# Autodesk Inventor assembly: FlexCouplerAssembly
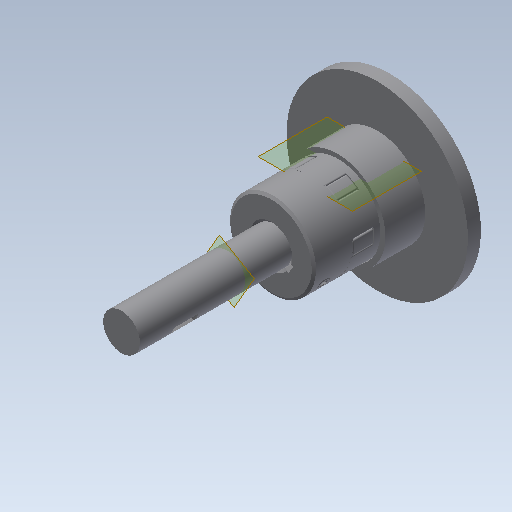
[picture p0: Inventor's stored thumbnail of the model, 512x512]
Saved by Autodesk Inventor 2021 (Build 250183000, 183)
## iProperties
Created: 2020-09-19
Part Number: FlexCouplerAssembly
Document SubType Name: Assembly
Designer: PhotonUser
Quantity: 1
Author: PhotonUser
## Documents named in this file (6)
- D:\PhotonUser\Downloads\Assembly Files-20201011T184130Z-001\Assembly Files\FlexCouplerAssembly.iam
- D:\PhotonUser\Downloads\Assembly Files-20201011T184130Z-001\Assembly Files\6408K139_FLEXIBLE SHAFT COUPLING ORIGINAL.ipt
- D:\PhotonUser\Downloads\Assembly Files-20201011T184130Z-001\Assembly Files\6408K139_FLEXIBLE SHAFT COUPLING.ipt
- D:\PhotonUser\Downloads\Assembly Files-20201011T184130Z-001\Assembly Files\6408K740_FLEXIBLE SHAFT RUBBER SPACER.ipt
- D:\PhotonUser\Downloads\Assembly Files-20201011T184130Z-001\Assembly Files\MotorFlexHub.ipt
- D:\PhotonUser\Downloads\Assembly Files-20201011T184130Z-001\Assembly Files\MotorShaft.ipt
## Components (5 placed, 5 different names)
1. 6408K139_FLEXIBLE SHAFT COUPLING ORIGINAL:1 — Insert:1, Mate:1, Mate:7, Mate:8
2. 6408K139_FLEXIBLE SHAFT COUPLING:1 — Mate:2, Mate:3, Mate:4, Mate:5, Mate:6, Insert:2
3. 6408K740_FLEXIBLE SHAFT RUBBER SPACER:1 — Insert:1, Mate:1, Mate:2, Mate:3, Mate:4, Mate:9
4. MotorFlexHub:1 — Mate:5, Mate:6, Insert:2
5. MotorShaft:1 — Mate:7, Mate:8, Mate:9
## Relationships (11: Mate 9, Insert 2)
- Insert:1: 6408K139_FLEXIBLE SHAFT COUPLING ORIGINAL:1 ↔ 6408K740_FLEXIBLE SHAFT RUBBER SPACER:1
- Mate:1: 6408K139_FLEXIBLE SHAFT COUPLING ORIGINAL:1 ↔ 6408K740_FLEXIBLE SHAFT RUBBER SPACER:1
- Mate:2: 6408K139_FLEXIBLE SHAFT COUPLING:1 ↔ 6408K740_FLEXIBLE SHAFT RUBBER SPACER:1
- Mate:3: 6408K139_FLEXIBLE SHAFT COUPLING:1 ↔ 6408K740_FLEXIBLE SHAFT RUBBER SPACER:1
- Mate:4: 6408K139_FLEXIBLE SHAFT COUPLING:1 ↔ 6408K740_FLEXIBLE SHAFT RUBBER SPACER:1
- Mate:5: 6408K139_FLEXIBLE SHAFT COUPLING:1 ↔ MotorFlexHub:1
- Mate:6: 6408K139_FLEXIBLE SHAFT COUPLING:1 ↔ MotorFlexHub:1
- Insert:2: 6408K139_FLEXIBLE SHAFT COUPLING:1 ↔ MotorFlexHub:1
- Mate:7: 6408K139_FLEXIBLE SHAFT COUPLING ORIGINAL:1 ↔ MotorShaft:1
- Mate:8: 6408K139_FLEXIBLE SHAFT COUPLING ORIGINAL:1 ↔ MotorShaft:1
- Mate:9: 6408K740_FLEXIBLE SHAFT RUBBER SPACER:1 ↔ MotorShaft:1
